# Autodesk Inventor assembly: Duck Carousel
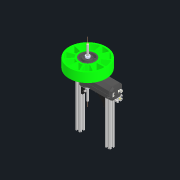
[picture p0: Inventor's stored thumbnail of the model, 180x180]
Saved by Autodesk Inventor 2022 (Build 260153000, 153)
## iProperties
Created: 2021-10-09
Part Number: Duck Carousel
Document SubType Name: Assembly
Designer: zehrab
Author: zehrab
## Documents named in this file (12)
- C:\Users\divid\Documents\GitHub\ComputerAidedDesign\2021-22\FTC\#13822 Robovikes\Duck Carousel\Duck Carousel.iam
- C:\Users\divid\Documents\GitHub\ComputerAidedDesign\2021-22\FTC\#13822 Robovikes\Duck Carousel\REV-41-1349.ipt
- C:\Users\divid\Documents\GitHub\ComputerAidedDesign\2021-22\FTC\#13822 Robovikes\Duck Carousel\am-4538 4IN 5mm Hex Compliant Wheel.ipt
- C:\Users\divid\Documents\GitHub\ComputerAidedDesign\2021-22\FTC\#13822 Robovikes\Duck Carousel\Slim Shaft Collar - 10 Pack.ipt
- C:\Users\divid\Documents\GitHub\ComputerAidedDesign\2021-22\FTC\#13822 Robovikes\Duck Carousel\3mm Spacer - 16 Pack.ipt
- C:\Users\divid\Documents\GitHub\ComputerAidedDesign\2021-22\FTC\#13822 Robovikes\Duck Carousel\REV-41-1300.ipt
- C:\Users\divid\Documents\GitHub\ComputerAidedDesign\2021-22\FTC\#13822 Robovikes\Duck Carousel\REV-41-1433.ipt
- C:\Users\divid\Documents\GitHub\ComputerAidedDesign\2021-22\FTC\#13822 Robovikes\Duck Carousel\15mm Extrusion - 120mm - 90° Ends - 2 Pack.ipt
- C:\Users\divid\Documents\GitHub\ComputerAidedDesign\2021-22\FTC\#13822 Robovikes\Duck Carousel\M3 x 8mm Hex Cap Screws - 100 Pack.ipt
- C:\Users\divid\Documents\GitHub\ComputerAidedDesign\2021-22\FTC\#13822 Robovikes\Duck Carousel\M3 Nyloc Nuts - 100 Pack.ipt
- C:\Users\divid\Documents\GitHub\ComputerAidedDesign\2021-22\FTC\#13822 Robovikes\Duck Carousel\REV-41-1320.ipt
- C:\Users\divid\Documents\GitHub\ComputerAidedDesign\2021-22\FTC\#13822 Robovikes\Duck Carousel\REV-41-1123.ipt
## Components (29 placed, 11 different names)
1. REV-41-1349:1 — Mate:10, Mate:11, Mate:12, Mate:13, Mate:14, Mate:17, Mate:19, Mate:39, Mate:40
2. am-4538 4IN 5mm Hex Compliant Wheel:1 — Mate:12, Mate:15, Mate:16
3. Slim Shaft Collar - 10 Pack:1 — Mate:10, Angle:6, Mate:15
4. Slim Shaft Collar - 10 Pack:2 — Mate:11, Angle:6, Mate:41
5. 3mm Spacer - 16 Pack:1 — Mate:13, Mate:14, Mate:16, Mate:18
6. REV-41-1300:1 — Mate:17, Mate:18, Mate:20, Angle:8, Mate:22, Mate:24, Mate:25, Mate:26, Mate:27
7. REV-41-1433:1 — Mate:19, Mate:20, Angle:8, Mate:21, Mate:23, Mate:31, Mate:33, Mate:35, Mate:36, Mate:38
8. 15mm Extrusion - 120mm - 90° Ends - 2 Pack:1 — Mate:21, Mate:22, Flush:5, Symmetry:1, Mate:28, Mate:29, Mate:42, Angle:9, Flush:6, Mate:44, Mate:54, Mate:59, Flush:8, Mate:61, Mate:65, Angle:10, Angle:11
9. M3 x 8mm Hex Cap Screws - 100 Pack:1 — Flush:2, Mate:23, Mate:24
10. M3 x 8mm Hex Cap Screws - 100 Pack:2 — Flush:2, Flush:3, Mate:25
11. M3 x 8mm Hex Cap Screws - 100 Pack:3 — Flush:3, Flush:4, Mate:26
12. M3 x 8mm Hex Cap Screws - 100 Pack:4 — Flush:4, Mate:27
13. M3 x 8mm Hex Cap Screws - 100 Pack:5 — Mate:28, Mate:32, Mate:33, Mate:37
14. M3 x 8mm Hex Cap Screws - 100 Pack:6 — Mate:29, Mate:30, Mate:31, Mate:34
15. M3 Nyloc Nuts - 100 Pack:1 — Mate:34, Mate:35
16. M3 Nyloc Nuts - 100 Pack:2 — Mate:36, Mate:37
17. 3mm Spacer - 16 Pack:2 — Mate:38, Mate:39, Mate:40, Mate:41
18. 15mm Extrusion - 120mm - 90° Ends - 2 Pack:2 — Mate:42, Angle:9, Flush:6, Mate:43, Flush:7, Symmetry:2, Mate:52
19. REV-41-1320:1 — Mate:43, Mate:44, Mate:45, Mate:51, Mate:53, Mate:55, Mate:58
20. REV-41-1123:1 — Mate:52, Mate:53, Mate:56
21. M3 Nyloc Nuts - 100 Pack:3 — Mate:51, Mate:56
22. REV-41-1123:2 — Mate:54, Mate:55, Mate:57
23. M3 Nyloc Nuts - 100 Pack:4 — Mate:57, Mate:58
24. 15mm Extrusion - 120mm - 90° Ends - 2 Pack:3 — Mate:59, Flush:8, Mate:60, Mate:62
25. REV-41-1123:3 — Mate:60, Mate:64, Mate:67
26. REV-41-1320:2 — Mate:61, Mate:62, Mate:63, Mate:64, Mate:66, Mate:68, Mate:70
27. REV-41-1123:4 — Mate:65, Mate:66, Mate:69
28. M3 Nyloc Nuts - 100 Pack:5 — Mate:67, Mate:68
29. M3 Nyloc Nuts - 100 Pack:6 — Mate:69, Mate:70
## Relationships (70: Mate 56, Flush 7, Angle 5, Symmetry 2)
- Mate:10: REV-41-1349:1 ↔ Slim Shaft Collar - 10 Pack:1
- Mate:11: REV-41-1349:1 ↔ Slim Shaft Collar - 10 Pack:2
- Angle:6 (0 deg): Slim Shaft Collar - 10 Pack:1 ↔ Slim Shaft Collar - 10 Pack:2
- Mate:12: REV-41-1349:1 ↔ am-4538 4IN 5mm Hex Compliant Wheel:1
- Mate:13: REV-41-1349:1 ↔ 3mm Spacer - 16 Pack:1
- Mate:14: REV-41-1349:1 ↔ 3mm Spacer - 16 Pack:1
- Mate:15: am-4538 4IN 5mm Hex Compliant Wheel:1 ↔ Slim Shaft Collar - 10 Pack:1
- Mate:16: am-4538 4IN 5mm Hex Compliant Wheel:1 ↔ 3mm Spacer - 16 Pack:1
- Mate:17: REV-41-1349:1 ↔ REV-41-1300:1
- Mate:18: 3mm Spacer - 16 Pack:1 ↔ REV-41-1300:1
- Mate:19: REV-41-1349:1 ↔ REV-41-1433:1
- Mate:20: REV-41-1300:1 ↔ REV-41-1433:1
- Angle:8 (180 deg): REV-41-1300:1 ↔ REV-41-1433:1
- Mate:21: REV-41-1433:1 ↔ 15mm Extrusion - 120mm - 90° Ends - 2 Pack:1
- Mate:22: REV-41-1300:1 ↔ 15mm Extrusion - 120mm - 90° Ends - 2 Pack:1
- Flush:2: M3 x 8mm Hex Cap Screws - 100 Pack:1 ↔ M3 x 8mm Hex Cap Screws - 100 Pack:2
- Flush:3: M3 x 8mm Hex Cap Screws - 100 Pack:2 ↔ M3 x 8mm Hex Cap Screws - 100 Pack:3
- Flush:4: M3 x 8mm Hex Cap Screws - 100 Pack:3 ↔ M3 x 8mm Hex Cap Screws - 100 Pack:4
- Mate:23: REV-41-1433:1 ↔ M3 x 8mm Hex Cap Screws - 100 Pack:1
- Mate:24: REV-41-1300:1 ↔ M3 x 8mm Hex Cap Screws - 100 Pack:1
- Mate:25: REV-41-1300:1 ↔ M3 x 8mm Hex Cap Screws - 100 Pack:2
- Mate:26: REV-41-1300:1 ↔ M3 x 8mm Hex Cap Screws - 100 Pack:3
- Mate:27: REV-41-1300:1 ↔ M3 x 8mm Hex Cap Screws - 100 Pack:4
- Flush:5: 15mm Extrusion - 120mm - 90° Ends - 2 Pack:1
- Symmetry:1: 15mm Extrusion - 120mm - 90° Ends - 2 Pack:1
- Mate:28: 15mm Extrusion - 120mm - 90° Ends - 2 Pack:1 ↔ M3 x 8mm Hex Cap Screws - 100 Pack:5
- Mate:29: 15mm Extrusion - 120mm - 90° Ends - 2 Pack:1 ↔ M3 x 8mm Hex Cap Screws - 100 Pack:6
- Mate:30: M3 x 8mm Hex Cap Screws - 100 Pack:6
- Mate:31: REV-41-1433:1 ↔ M3 x 8mm Hex Cap Screws - 100 Pack:6
- Mate:32: M3 x 8mm Hex Cap Screws - 100 Pack:5
- Mate:33: REV-41-1433:1 ↔ M3 x 8mm Hex Cap Screws - 100 Pack:5
- Mate:34: M3 x 8mm Hex Cap Screws - 100 Pack:6 ↔ M3 Nyloc Nuts - 100 Pack:1
- Mate:35: REV-41-1433:1 ↔ M3 Nyloc Nuts - 100 Pack:1
- Mate:36: REV-41-1433:1 ↔ M3 Nyloc Nuts - 100 Pack:2
- Mate:37: M3 x 8mm Hex Cap Screws - 100 Pack:5 ↔ M3 Nyloc Nuts - 100 Pack:2
- Mate:38: REV-41-1433:1 ↔ 3mm Spacer - 16 Pack:2
- Mate:39: REV-41-1349:1 ↔ 3mm Spacer - 16 Pack:2
- Mate:40: REV-41-1349:1 ↔ 3mm Spacer - 16 Pack:2
- Mate:41: Slim Shaft Collar - 10 Pack:2 ↔ 3mm Spacer - 16 Pack:2
- Mate:42: 15mm Extrusion - 120mm - 90° Ends - 2 Pack:1 ↔ 15mm Extrusion - 120mm - 90° Ends - 2 Pack:2
- Angle:9 (0 deg): 15mm Extrusion - 120mm - 90° Ends - 2 Pack:1 ↔ 15mm Extrusion - 120mm - 90° Ends - 2 Pack:2
- Flush:6: 15mm Extrusion - 120mm - 90° Ends - 2 Pack:1 ↔ 15mm Extrusion - 120mm - 90° Ends - 2 Pack:2
- Mate:43: 15mm Extrusion - 120mm - 90° Ends - 2 Pack:2 ↔ REV-41-1320:1
- Mate:44: 15mm Extrusion - 120mm - 90° Ends - 2 Pack:1 ↔ REV-41-1320:1
- Flush:7: 15mm Extrusion - 120mm - 90° Ends - 2 Pack:2
- Symmetry:2: 15mm Extrusion - 120mm - 90° Ends - 2 Pack:2
- Mate:45: REV-41-1320:1
- Mate:51: REV-41-1320:1 ↔ M3 Nyloc Nuts - 100 Pack:3
- Mate:52: 15mm Extrusion - 120mm - 90° Ends - 2 Pack:2 ↔ REV-41-1123:1
- Mate:53: REV-41-1320:1 ↔ REV-41-1123:1
- Mate:54: 15mm Extrusion - 120mm - 90° Ends - 2 Pack:1 ↔ REV-41-1123:2
- Mate:55: REV-41-1320:1 ↔ REV-41-1123:2
- Mate:56: REV-41-1123:1 ↔ M3 Nyloc Nuts - 100 Pack:3
- Mate:57: REV-41-1123:2 ↔ M3 Nyloc Nuts - 100 Pack:4
- Mate:58: REV-41-1320:1 ↔ M3 Nyloc Nuts - 100 Pack:4
- Mate:59: 15mm Extrusion - 120mm - 90° Ends - 2 Pack:1 ↔ 15mm Extrusion - 120mm - 90° Ends - 2 Pack:3
- Flush:8: 15mm Extrusion - 120mm - 90° Ends - 2 Pack:1 ↔ 15mm Extrusion - 120mm - 90° Ends - 2 Pack:3
- Mate:60: 15mm Extrusion - 120mm - 90° Ends - 2 Pack:3 ↔ REV-41-1123:3
- Mate:61: 15mm Extrusion - 120mm - 90° Ends - 2 Pack:1 ↔ REV-41-1320:2
- Mate:62: 15mm Extrusion - 120mm - 90° Ends - 2 Pack:3 ↔ REV-41-1320:2
- Mate:63: REV-41-1320:2
- Mate:64: REV-41-1123:3 ↔ REV-41-1320:2
- Mate:65: 15mm Extrusion - 120mm - 90° Ends - 2 Pack:1 ↔ REV-41-1123:4
- Mate:66: REV-41-1320:2 ↔ REV-41-1123:4
- Mate:67: REV-41-1123:3 ↔ M3 Nyloc Nuts - 100 Pack:5
- Mate:68: REV-41-1320:2 ↔ M3 Nyloc Nuts - 100 Pack:5
- Mate:69: REV-41-1123:4 ↔ M3 Nyloc Nuts - 100 Pack:6
- Mate:70: REV-41-1320:2 ↔ M3 Nyloc Nuts - 100 Pack:6
- Angle:10 (0 deg): 15mm Extrusion - 120mm - 90° Ends - 2 Pack:1
- Angle:11 (0 deg): 15mm Extrusion - 120mm - 90° Ends - 2 Pack:1
